# Autodesk Inventor assembly: Kompetente Baugruppe
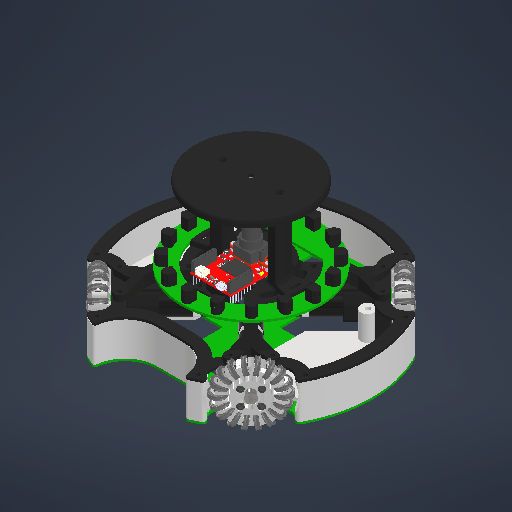
[picture p0: Inventor's stored thumbnail of the model, 512x512]
Saved by Autodesk Inventor 2025.3 (Build 293356000, 356)
## iProperties
Created: 2025-05-27
Part Number: Kompetente Baugruppe
Document SubType Name: Assembly
Designer: theod
Author: theod
## Documents named in this file (7)
- C:\Users\theod\Desktop\Team Mathimazierer v2025\Kompetente Baugruppe.iam
- C:\Users\theod\Desktop\Team Mathimazierer v2025\Antrieb final.iam
- C:\Users\theod\Desktop\Team Mathimazierer v2025\Oberer Teil.iam
- C:\Users\theod\Desktop\Team Mathimazierer v2025\Wände.ipt
- C:\Users\theod\Desktop\Team Mathimazierer v2025\Ballkuhle.ipt
- C:\Users\theod\Nextcloud\Inventor\2vs2 LWL Int. 2025\Wand hinten.ipt
- C:\Users\theod\Desktop\Team Mathimazierer v2025\Boden WM.ipt
## Components (10 placed, 6 different names)
1. Oberer Teil:1 [sub-assembly] — Passend:9, Passend:10, Einfügen:11, Einfügen:12, Passend:11, Passend:12, Passend:13, Passend:14, Passend:15, Passend:16
2. Wände:1
3. Ballkuhle:1 — Passend:9, Passend:10, Passend:18, Passend:19, Passend:26
4. Wände:2 — Passend:11, Passend:12, Passend:13, Passend:17
5. Wand hinten:1 — Passend:14, Passend:15, Passend:16
6. Boden WM:1 — Passend:17, Passend:18, Passend:19, Passend:26
7. Antrieb final:1 [sub-assembly] — Einfügen:11, Einfügen:12
8. Antrieb final:2 [sub-assembly]
9. Antrieb final:3 [sub-assembly]
10. Antrieb final:4 [sub-assembly]
## Component patterns: (4 elements, first: Antrieb final:1)
## Relationships (14: Mate 12, Insert 2)
- Passend:9 [Mate]: Oberer Teil:1 ↔ Ballkuhle:1
- Passend:10 [Mate]: Oberer Teil:1 ↔ Ballkuhle:1
- Einfügen:11 [Insert]: Oberer Teil:1 ↔ Antrieb final:1
- Einfügen:12 [Insert]: Oberer Teil:1 ↔ Antrieb final:1
- Passend:11 [Mate]: Oberer Teil:1 ↔ Wände:2
- Passend:12 [Mate]: Oberer Teil:1 ↔ Wände:2
- Passend:13 [Mate]: Oberer Teil:1 ↔ Wände:2
- Passend:14 [Mate]: Oberer Teil:1 ↔ Wand hinten:1
- Passend:15 [Mate]: Oberer Teil:1 ↔ Wand hinten:1
- Passend:16 [Mate]: Oberer Teil:1 ↔ Wand hinten:1
- Passend:17 [Mate]: Wände:2 ↔ Boden WM:1
- Passend:18 [Mate]: Ballkuhle:1 ↔ Boden WM:1
- Passend:19 [Mate]: Ballkuhle:1 ↔ Boden WM:1
- Passend:26 [Mate]: Ballkuhle:1 ↔ Boden WM:1
